# Autodesk Inventor assembly: serwo
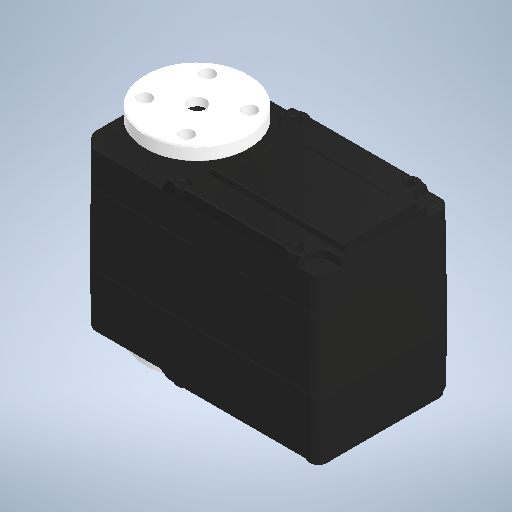
[picture p0: Inventor's stored thumbnail of the model, 512x512]
Saved by Autodesk Inventor 2025.3 (Build 293356000, 356)
## iProperties
Created: 2026-05-08
Part Number: serwo
Document SubType Name: Assembly
Designer: ksawe
Author: ksawe
## Documents named in this file (3)
- C:\Users\ksawe\OneDrive\Pulpit\Exomy v1\wersja3\serwo.iam
- C:\Users\ksawe\OneDrive\Pulpit\Exomy v1\wersja2\ST3215\ST3215\ST3215.iam
- C:\Users\ksawe\OneDrive\Pulpit\Exomy v1\wersja2\ST3215\ST3215\金属舵盘（驱动） v2.ipt
## Components (2 placed, 2 different names)
1. ST3215:1 [sub-assembly] — Rotational:1
2. 金属舵盘（驱动） v2:1 — Rotational:1
## Relationships (1: RevoluteJoint 1)
- Rotational:1 [RevoluteJoint]: ST3215:1 ↔ 金属舵盘（驱动） v2:1
